# Autodesk Inventor assembly: stopper
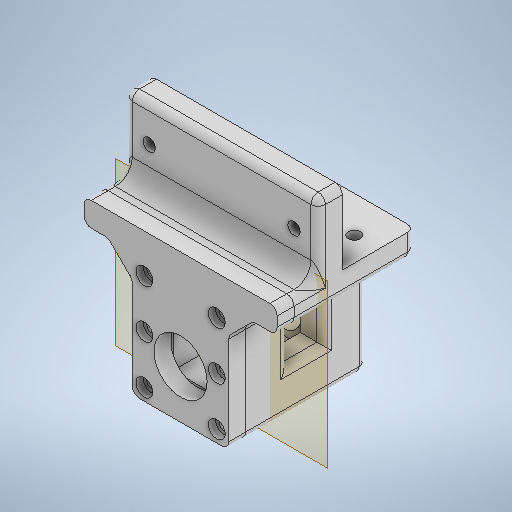
[picture p0: Inventor's stored thumbnail of the model, 512x512]
Saved by Autodesk Inventor 2026.1 (Build 301233000, 233)
## iProperties
Created: 2026-05-21
Part Number: stopper
Document SubType Name: Assembly
Designer: chris
Author: chris
## Documents named in this file (3)
- C:\Users\chris\Documents\yonsei\4-1\창의제품설계\design\CLOSE_hardware\04그리퍼\stopper\stopper.iam
- C:\Users\chris\Documents\yonsei\4-1\창의제품설계\design\CLOSE_hardware\04그리퍼\stopper\stopper_motor_bracket.ipt
- C:\Users\chris\Documents\yonsei\4-1\창의제품설계\design\CLOSE_hardware\04그리퍼\stopper\stopper_motor_bracket_cover.ipt
## Components (2 placed, 2 different names)
1. stopper_motor_bracket:1 — Mate:1, Flush:1, Flush:2
2. stopper_motor_bracket_cover:1 — Mate:1, Flush:1, Flush:2
## Relationships (3: Flush 2, Mate 1)
- Mate:1: stopper_motor_bracket:1 ↔ stopper_motor_bracket_cover:1
- Flush:1: stopper_motor_bracket:1 ↔ stopper_motor_bracket_cover:1
- Flush:2: stopper_motor_bracket:1 ↔ stopper_motor_bracket_cover:1
